# Autodesk Inventor assembly: Tendeur
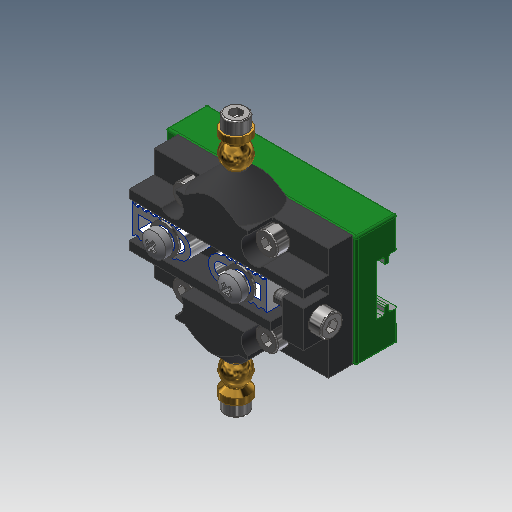
[picture p0: Inventor's stored thumbnail of the model, 512x512]
Saved by Autodesk Inventor 2017 (Build 210142000, 142)
## iProperties
Company: FABLAB Frenchmakers
Part Number: Tendeur
Material: Générique
Document SubType Name: Assembly
Designer: FABLAB Frenchmakers
Mass: 32.7451 g
Surface Area: 136.04 cm^2
Volume: 21.17 cm^3
Density: 1.54677 g/cm^3
Project: 1420 Vauban 3D XL
Catalog Web Link: http://frenchmakers.com/
Stock Number: 1420-12-00
## Documents named in this file (9)
- W:\Professionnel\Conception FABLAB\1420-Vauban 3D XL\1420-12 Guidage\1420-12-00 Tendeur.iam
- W:\Professionnel\Conception FABLAB\1420-Vauban 3D XL\1420-12 Guidage\1420-12-05 Tendeur.ipt
- W:\Professionnel\Conception FABLAB\1420-Vauban 3D XL\1420-12 Guidage\1420-12-06 Contre rondelle.ipt
- W:\Professionnel\Conception FABLAB\1420-Vauban 3D XL\1420-12 Guidage\1420-12-04 Platine.ipt
- W:\Professionnel\Conception FABLAB\1420-Vauban 3D XL\1420-12 Guidage\1420-12-02 Cage a bille.ipt
- W:\Professionnel\Conception FABLAB\1420-Vauban 3D XL\1420-90 Centre de contenu\fr-FR\DIN 7985 (H)\DIN 7985 (H) - M3x12-H.ipt
- W:\Professionnel\Conception FABLAB\1420-Vauban 3D XL\1420-90 Centre de contenu\fr-FR\DIN 125-1  A\DIN 125 - A 3,2.ipt
- W:\Professionnel\Conception FABLAB\1420-Vauban 3D XL\1420-90 Centre de contenu\fr-FR\ANSI B18.3.1M(1)\ANSI B18.3.1M - M3x0,5 x 10(2).ipt
- W:\Professionnel\Conception FABLAB\1420-Vauban 3D XL\1420-10 Bras\1420-10-03 Rotule avec meplat.ipt
## Components (19 placed, 8 different names)
1. 1420-12-04 Platine:1 — Placage:2, Placage:3, Placage:4, Placage:5, Placage:6, Placage:7, Placage:8, Placage:17, Placage:18, Placage:19, Placage:20, Placage:21, Placage:22, Placage:23, Placage:24, Placage:25, Placage:30, Placage:31
2. 1420-12-05 Tendeur:1 — Affleurement:4, Placage:15, Placage:32
3. 1420-12-05 Tendeur:2 — Affleurement:4, Placage:12, Placage:16
4. 1420-12-06 Contre rondelle:1 — Placage:6, Placage:10
5. 1420-12-06 Contre rondelle:2 — Placage:5, Placage:9, Placage:14
6. 1420-12-02 Cage a bille:1 — Placage:2, Placage:3, Placage:4
7. DIN 7985 (H) M3x12-H:1 — Placage:8, Affleurement:5, Placage:10, Placage:11, Placage:16
8. DIN 7985 (H) M3x12-H:2 — Placage:7, Affleurement:5, Placage:9, Placage:13, Placage:15
9. DIN 125-1 A A 3,2:1 — Affleurement:6, Placage:13, Placage:14
10. DIN 125-1 A A 3,2:2 — Affleurement:6, Placage:11, Placage:12
11. Vis à tête percée - Métrique M3x0,5 x 10:1 — Affleurement:7, Affleurement:8, Placage:17
12. Vis à tête percée - Métrique M3x0,5 x 10:2 — Affleurement:7, Placage:18, Placage:21
13. Vis à tête percée - Métrique M3x0,5 x 10:3 — Affleurement:8, Affleurement:9, Placage:19
14. Vis à tête percée - Métrique M3x0,5 x 10:4 — Affleurement:9, Placage:20
15. 1420-10-03 Rotule avec meplat:1 — Placage:23, Placage:24, Placage:28, Placage:29
16. 1420-10-03 Rotule avec meplat:2 — Placage:22, Placage:25, Placage:26, Placage:27
17. Vis à tête percée - Métrique M3x0,5 x 10:5 — Placage:28, Placage:29
18. Vis à tête percée - Métrique M3x0,5 x 10:6 — Placage:26, Placage:27
19. Vis à tête percée - Métrique M3x0,5 x 10:7 — Placage:30, Placage:31, Placage:32
## Relationships (43: Mate 32, Flush 9, Angle 2)
- [Flush]: 1420-12-04 Platine:1
- [Flush]: 1420-12-04 Platine:1
- [Flush]: 1420-12-04 Platine:1
- Affleurement:4 [Flush]: 1420-12-05 Tendeur:1 ↔ 1420-12-05 Tendeur:2
- [Mate]: 1420-12-04 Platine:1 ↔ 1420-12-05 Tendeur:2
- [Angle] (180 deg): 1420-12-04 Platine:1 ↔ 1420-12-05 Tendeur:2
- [Angle] (0 deg): 1420-12-04 Platine:1 ↔ 1420-12-05 Tendeur:1
- Placage:2 [Mate]: 1420-12-04 Platine:1 ↔ 1420-12-02 Cage a bille:1
- Placage:3 [Mate]: 1420-12-04 Platine:1 ↔ 1420-12-02 Cage a bille:1
- Placage:4 [Mate]: 1420-12-04 Platine:1 ↔ 1420-12-02 Cage a bille:1
- Placage:5 [Mate]: 1420-12-04 Platine:1 ↔ 1420-12-06 Contre rondelle:2
- Placage:6 [Mate]: 1420-12-04 Platine:1 ↔ 1420-12-06 Contre rondelle:1
- Placage:7 [Mate]: 1420-12-04 Platine:1 ↔ DIN 7985 (H) M3x12-H:2
- Placage:8 [Mate]: 1420-12-04 Platine:1 ↔ DIN 7985 (H) M3x12-H:1
- Affleurement:5 [Flush]: DIN 7985 (H) M3x12-H:1 ↔ DIN 7985 (H) M3x12-H:2
- Placage:9 [Mate]: 1420-12-06 Contre rondelle:2 ↔ DIN 7985 (H) M3x12-H:2
- Placage:10 [Mate]: 1420-12-06 Contre rondelle:1 ↔ DIN 7985 (H) M3x12-H:1
- Affleurement:6 [Flush]: DIN 125-1 A A 3,2:1 ↔ DIN 125-1 A A 3,2:2
- Placage:11 [Mate]: DIN 7985 (H) M3x12-H:1 ↔ DIN 125-1 A A 3,2:2
- Placage:12 [Mate]: 1420-12-05 Tendeur:2 ↔ DIN 125-1 A A 3,2:2
- Placage:13 [Mate]: DIN 7985 (H) M3x12-H:2 ↔ DIN 125-1 A A 3,2:1
- Placage:14 [Mate]: 1420-12-06 Contre rondelle:2 ↔ DIN 125-1 A A 3,2:1
- Placage:15 [Mate]: 1420-12-05 Tendeur:1 ↔ DIN 7985 (H) M3x12-H:2
- Placage:16 [Mate]: 1420-12-05 Tendeur:2 ↔ DIN 7985 (H) M3x12-H:1
- Affleurement:7 [Flush]: Vis à tête percée - Métrique M3x0,5 x 10:1 ↔ Vis à tête percée - Métrique M3x0,5 x 10:2
- Affleurement:8 [Flush]: Vis à tête percée - Métrique M3x0,5 x 10:1 ↔ Vis à tête percée - Métrique M3x0,5 x 10:3
- Affleurement:9 [Flush]: Vis à tête percée - Métrique M3x0,5 x 10:3 ↔ Vis à tête percée - Métrique M3x0,5 x 10:4
- Placage:17 [Mate]: 1420-12-04 Platine:1 ↔ Vis à tête percée - Métrique M3x0,5 x 10:1
- Placage:18 [Mate]: 1420-12-04 Platine:1 ↔ Vis à tête percée - Métrique M3x0,5 x 10:2
- Placage:19 [Mate]: 1420-12-04 Platine:1 ↔ Vis à tête percée - Métrique M3x0,5 x 10:3
- Placage:20 [Mate]: 1420-12-04 Platine:1 ↔ Vis à tête percée - Métrique M3x0,5 x 10:4
- Placage:21 [Mate]: 1420-12-04 Platine:1 ↔ Vis à tête percée - Métrique M3x0,5 x 10:2
- Placage:22 [Mate]: 1420-12-04 Platine:1 ↔ 1420-10-03 Rotule avec meplat:2
- Placage:23 [Mate]: 1420-12-04 Platine:1 ↔ 1420-10-03 Rotule avec meplat:1
- Placage:24 [Mate]: 1420-12-04 Platine:1 ↔ 1420-10-03 Rotule avec meplat:1
- Placage:25 [Mate]: 1420-12-04 Platine:1 ↔ 1420-10-03 Rotule avec meplat:2
- Placage:26 [Mate]: 1420-10-03 Rotule avec meplat:2 ↔ Vis à tête percée - Métrique M3x0,5 x 10:6
- Placage:27 [Mate]: 1420-10-03 Rotule avec meplat:2 ↔ Vis à tête percée - Métrique M3x0,5 x 10:6
- Placage:28 [Mate]: 1420-10-03 Rotule avec meplat:1 ↔ Vis à tête percée - Métrique M3x0,5 x 10:5
- Placage:29 [Mate]: 1420-10-03 Rotule avec meplat:1 ↔ Vis à tête percée - Métrique M3x0,5 x 10:5
- Placage:30 [Mate]: 1420-12-04 Platine:1 ↔ Vis à tête percée - Métrique M3x0,5 x 10:7
- Placage:31 [Mate] (0.5 mm): 1420-12-04 Platine:1 ↔ Vis à tête percée - Métrique M3x0,5 x 10:7
- Placage:32 [Mate]: 1420-12-05 Tendeur:1 ↔ Vis à tête percée - Métrique M3x0,5 x 10:7
